# Autodesk Inventor assembly: Auspressrolle_befaesstigung
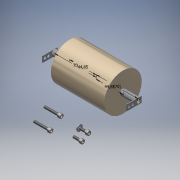
[picture p0: Inventor's stored thumbnail of the model, 180x180]
Saved by Autodesk Inventor 2018 (Build 220112000, 112)
## iProperties
Created: 2018-01-12
Part Number: Auspressrolle_befaesstigung
Material: Generisch
Document SubType Name: Assembly
Designer: Julian
Author: Julian
## Documents named in this file (8)
- C:\Users\Julian\Desktop\Schule\5AHME\Diplomarbeit\Git\fuettr_prototype\Mechanical\Inventorskizzen\Auspressrolle_befaesstigung.iam
- C:\Users\Julian\Desktop\Schule\5AHME\Diplomarbeit\Git\fuettr_prototype\Mechanical\Inventorskizzen\Auspressrolle.ipt
- C:\Users\Julian\Desktop\Schule\5AHME\Diplomarbeit\Git\fuettr_prototype\Mechanical\Inventorskizzen\Verbindungsstück_Rolle.ipt
- C:\Users\Julian\Desktop\Schule\5AHME\Diplomarbeit\Git\fuettr_prototype\Mechanical\Inventorskizzen\Kunststoffrolle_antrieb.ipt
- C:\Users\Julian\Documents\Inventor\Content Center Files\R2018\de-DE\DIN 471(1)\DIN 471 - 8x0,8.ipt
- C:\Users\Julian\Documents\Inventor\Content Center Files\R2018\de-DE\ISO 4762(1)\DIN EN ISO 4762 - M4 x 12.ipt
- C:\Users\Julian\Documents\Inventor\Content Center Files\R2018\de-DE\ISO 4762(1)\DIN EN ISO 4762 - M4 x 25.ipt
- C:\Users\Julian\Documents\Inventor\Content Center Files\R2018\de-DE\DIN 988(1)\DIN 988 - S5 x 10.ipt
## Components (11 placed, 7 different names)
1. Auspressrolle:1 — Starr:1, Starr:2, Passend:1, Fluchtend:1, Starr:4, Starr:3
2. Verbindungsstück_Rolle:1 — Starr:1
3. Verbindungsstück_Rolle:2 — Starr:2
4. Kunststoffrolle_antrieb:1 — Passend:1, Fluchtend:1
5. DIN 471 8x0,8:1 — Starr:3
6. DIN 471 8x0,8:2 — Starr:4
7. DIN EN ISO 4762 M4 x 12:1 — Passend:2
8. DIN EN ISO 4762 M4 x 12:2
9. DIN EN ISO 4762 M4 x 25:1
10. DIN EN ISO 4762 M4 x 25:2
11. DIN 988 S5 x 10:1 — Passend:2
## Relationships (7: WeldJoint 4, Mate 2, Flush 1)
- Starr:1 [WeldJoint]: Auspressrolle:1 ↔ Verbindungsstück_Rolle:1
- Starr:2 [WeldJoint]: Auspressrolle:1 ↔ Verbindungsstück_Rolle:2
- Passend:1 [Mate]: Auspressrolle:1 ↔ Kunststoffrolle_antrieb:1
- Fluchtend:1 [Flush]: Auspressrolle:1 ↔ Kunststoffrolle_antrieb:1
- Starr:4 [WeldJoint]: Auspressrolle:1 ↔ DIN 471 8x0,8:2
- Starr:3 [WeldJoint]: Auspressrolle:1 ↔ DIN 471 8x0,8:1
- Passend:2 [Mate]: DIN EN ISO 4762 M4 x 12:1 ↔ DIN 988 S5 x 10:1
